# Autodesk Inventor assembly: B_Legs0
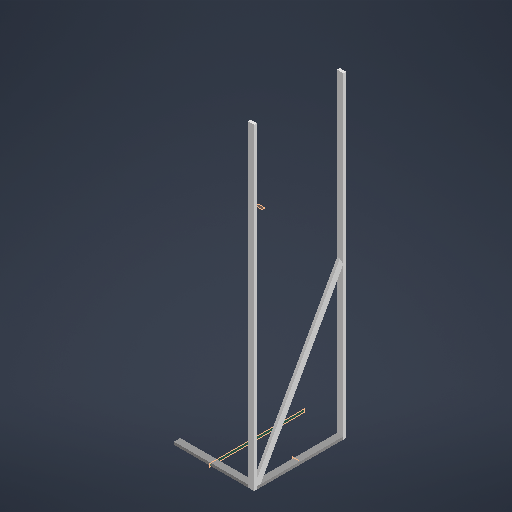
[picture p0: Inventor's stored thumbnail of the model, 512x512]
Saved by Autodesk Inventor 2026 (Build 300175000, 175)
## iProperties
Created: 2024-09-19
Part Number: B_Legs0
Document SubType Name: Assembly
Designer: User
Author: User
## Documents named in this file (5)
- C:\Users\trott\Documents\UofSC-ASME-Tiger-Burn-Design-2025\CAD\Legs\Front Leg\F_Leg.iam
- C:\Users\trott\Documents\UofSC-ASME-Tiger-Burn-Design-2025\CAD\Legs\Front Leg\2x4x42.ipt
- C:\Users\trott\Documents\UofSC-ASME-Tiger-Burn-Design-2025\CAD\Legs\Front Leg\2x4x48.ipt
- C:\Users\trott\Documents\UofSC-ASME-Tiger-Burn-Design-2025\CAD\Legs\Front Leg\2x4x176.ipt
- C:\Users\trott\Documents\UofSC-ASME-Tiger-Burn-Design-2025\CAD\Legs\Front Leg\S_2x4x98.925.ipt
## Components (5 placed, 4 different names)
1. 2x4x176:1 — Flush:27, Mate:18, Flush:28, Mate:19, Flush:30, Flush:39
2. 2x4x42:5 — Flush:27, Mate:18, Flush:28, Flush:29
3. 2x4x48:5 — Flush:29, Mate:19, Flush:30, Flush:31, Flush:34, Mate:23, Mate:24, Flush:40, Flush:41
4. S_2x4x98.925:1 — Mate:23, Flush:39
5. 2x4x176:2 — Mate:24, Flush:40, Flush:41
## Relationships (13: Flush 9, Mate 4)
- Flush:27: 2x4x176:1 ↔ 2x4x42:5
- Mate:18: 2x4x176:1 ↔ 2x4x42:5
- Flush:28: 2x4x176:1 ↔ 2x4x42:5
- Flush:29: 2x4x42:5 ↔ 2x4x48:5
- Mate:19: 2x4x176:1 ↔ 2x4x48:5
- Flush:30: 2x4x176:1 ↔ 2x4x48:5
- Flush:31 (520.7 mm): 2x4x48:5
- Flush:34 (-609.6 mm): 2x4x48:5
- Mate:23: 2x4x48:5 ↔ S_2x4x98.925:1
- Flush:39: 2x4x176:1 ↔ S_2x4x98.925:1
- Mate:24: 2x4x48:5 ↔ 2x4x176:2
- Flush:40: 2x4x48:5 ↔ 2x4x176:2
- Flush:41: 2x4x48:5 ↔ 2x4x176:2
